# Autodesk Inventor assembly: anschluss_daten
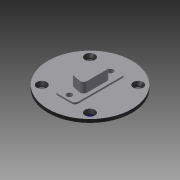
[picture p0: Inventor's stored thumbnail of the model, 180x180]
Saved by Autodesk Inventor 2015 (Build 190159000, 159)
## iProperties
Created: 2018-04-03
Part Number: anschluss_daten
Document SubType Name: Assembly
Designer: wepet
Author: wepet
## Documents named in this file (3)
- C:\workspace\robosax\licht\Zusatzelemente\anschluss_daten.iam
- C:\workspace\robosax\licht\Zusatzelemente\anschluss_daten_1.ipt
- C:\workspace\robosax\licht\Zusatzelemente\anschluss_daten_2.ipt
## Components (2 placed, 2 different names)
1. anschluss_daten_1:1 — Drehbar:1, Drehbar:2, Passend:1
2. anschluss_daten_2:1 — Drehbar:1, Drehbar:2, Passend:2, Fluchtend:1
## Relationships (5: RevoluteJoint 2, Mate 2, Flush 1)
- Drehbar:1 [RevoluteJoint]: anschluss_daten_1:1 ↔ anschluss_daten_2:1
- Drehbar:2 [RevoluteJoint]: anschluss_daten_1:1 ↔ anschluss_daten_2:1
- Passend:1 [Mate]: anschluss_daten_1:1
- Passend:2 [Mate] (-4.18 mm): anschluss_daten_2:1
- Fluchtend:1 [Flush] (-15.405 mm): anschluss_daten_2:1
